# Autodesk Inventor assembly: MSI-000
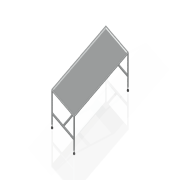
[picture p0: Inventor's stored thumbnail of the model, 180x180]
Saved by Autodesk Inventor 2020.3 (Build 243373000, 373)
## iProperties
Created: 2021-02-10
Part Number: MSI-000
Document SubType Name: Assembly
Designer: Adriano
Author: Adriano
## Documents named in this file (5)
- C:\Users\Adriano\Documents\Inventor\Mesa_Inox\MSI-000.iam
- C:\Users\Adriano\Documents\Inventor\Mesa_Inox\MSI-100.iam
- C:\Users\Adriano\Documents\Inventor\Mesa_Inox\MSI-001.ipt
- C:\Users\Adriano\Documents\Inventor\Mesa_Inox\ACAB_TUBO_40X40.ipt
- C:\Users\Adriano\Documents\Inventor\Mesa_Inox\PE_NIV_80.ipt
## Components (10 placed, 4 different names)
1. MSI-100:1 [sub-assembly] — Coincidência:1, Coincidência:2, Alinhamento:1, Coincidência:3, Alinhamento:2, Coincidência:6, Coincidência:7, Alinhamento:3, Alinhamento:4, Alinhamento:5, Coincidência:8, Alinhamento:6, Coincidência:9, Alinhamento:7, Coincidência:10, Alinhamento:8
2. MSI-001:1 — Coincidência:1, Coincidência:4, Coincidência:5
3. ACAB_TUBO_40X40:1 — Alinhamento:2, Coincidência:6, Coincidência:7, Inserir:1
4. PE_NIV_80:1 — Inserir:1
5. ACAB_TUBO_40X40:2 — Alinhamento:3, Alinhamento:5, Coincidência:8, Inserir:2
6. PE_NIV_80:2 — Inserir:2
7. ACAB_TUBO_40X40:3 — Alinhamento:4, Alinhamento:6, Coincidência:9, Inserir:3
8. PE_NIV_80:3 — Inserir:3
9. ACAB_TUBO_40X40:4 — Alinhamento:7, Coincidência:10, Alinhamento:8, Inserir:4
10. PE_NIV_80:4 — Inserir:4
## Relationships (22: Mate 10, Flush 8, Insert 4)
- Coincidência:1 [Mate]: MSI-100:1 ↔ MSI-001:1
- Coincidência:2 [Mate]: MSI-100:1
- Alinhamento:1 [Flush]: MSI-100:1
- Coincidência:3 [Mate]: MSI-100:1
- Coincidência:4 [Mate]: MSI-001:1
- Coincidência:5 [Mate]: MSI-001:1
- Alinhamento:2 [Flush]: MSI-100:1 ↔ ACAB_TUBO_40X40:1
- Coincidência:6 [Mate]: MSI-100:1 ↔ ACAB_TUBO_40X40:1
- Coincidência:7 [Mate]: MSI-100:1 ↔ ACAB_TUBO_40X40:1
- Alinhamento:3 [Flush]: MSI-100:1 ↔ ACAB_TUBO_40X40:2
- Alinhamento:4 [Flush]: MSI-100:1 ↔ ACAB_TUBO_40X40:3
- Alinhamento:5 [Flush]: MSI-100:1 ↔ ACAB_TUBO_40X40:2
- Coincidência:8 [Mate]: MSI-100:1 ↔ ACAB_TUBO_40X40:2
- Alinhamento:6 [Flush]: MSI-100:1 ↔ ACAB_TUBO_40X40:3
- Coincidência:9 [Mate]: MSI-100:1 ↔ ACAB_TUBO_40X40:3
- Alinhamento:7 [Flush]: MSI-100:1 ↔ ACAB_TUBO_40X40:4
- Coincidência:10 [Mate]: MSI-100:1 ↔ ACAB_TUBO_40X40:4
- Alinhamento:8 [Flush]: MSI-100:1 ↔ ACAB_TUBO_40X40:4
- Inserir:1: ACAB_TUBO_40X40:1 ↔ PE_NIV_80:1
- Inserir:2: ACAB_TUBO_40X40:2 ↔ PE_NIV_80:2
- Inserir:3: ACAB_TUBO_40X40:3 ↔ PE_NIV_80:3
- Inserir:4: ACAB_TUBO_40X40:4 ↔ PE_NIV_80:4
